# Autodesk Inventor assembly: liftpossible
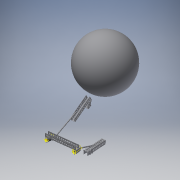
[picture p0: Inventor's stored thumbnail of the model, 180x180]
Saved by Autodesk Inventor 2016 (Build 200138000, 138)
## iProperties
Created: 2017-01-28
Part Number: liftpossible
Document SubType Name: Assembly
Designer: RoboticsUser
Author: RoboticsUser
## Documents named in this file (9)
- C:\Robotics\CAD\2016-17_CAD\liftpossible.iam
- C:\Robotics\CAD\2016-17_CAD\CapBall2.ipt
- C:\Robotics\CAD\COTSParts\Actobotics\585 parts\585450.ipt
- C:\Robotics\CAD\COTSParts\Actobotics\585 parts\585440.ipt
- C:\Robotics\CAD\COTSParts\Actobotics\585 parts\585404.ipt
- C:\Robotics\CAD\COTSParts\Actobotics\585 parts\585423.ipt
- C:\Robotics\CAD\COTSParts\Tetrix\Tetrix servo 180.ipt
- C:\Robotics\CAD\COTSParts\Tetrix\ptp_tetrix_servoframe_bracket.ipt
- C:\Robotics\CAD\COTSParts\Actobotics\585 parts\585454.ipt
## Components (20 placed, 8 different names)
1. CapBall2:1
2. 585450:1 — Insert:1, Insert:2, Insert:5, Insert:7, Insert:17
3. 585450:2 — Insert:9, Insert:10, Insert:11, Insert:12, Insert:18
4. 585440:1 — Insert:3, Insert:4, Insert:6, Insert:8
5. 585440:2 — Insert:13, Insert:14, Insert:15, Insert:16
6. 585404:1 — Insert:1, Insert:4
7. 585404:2 — Insert:2, Insert:3
8. 585423:1 — Insert:18, Insert:20
9. 585423:2 — Insert:17, Insert:19
10. 585404:3 — Insert:7, Insert:8
11. 585404:4 — Insert:5, Insert:6
12. 585404:5 — Insert:12, Insert:14
13. 585404:6 — Insert:9, Insert:15
14. 585404:7 — Insert:10, Insert:16
15. 585404:8 — Insert:11, Insert:13
16. Tetrix servo 180:1 — Insert:19, Mate:3, Mate:4, Flush:2
17. Tetrix servo 180:2 — Insert:20, Mate:1, Mate:2, Flush:1
18. ptp_tetrix_servoframe_bracket:1 — Mate:1, Mate:2, Flush:1, Mate:6, Flush:5, Flush:6
19. ptp_tetrix_servoframe_bracket:2 — Mate:3, Mate:4, Flush:2, Flush:3, Flush:4, Mate:5
20. 585454:1 — Flush:3, Flush:4, Mate:5, Mate:6, Flush:5, Flush:6
## Relationships (32: Insert 20, Mate 6, Flush 6)
- Insert:1: 585450:1 ↔ 585404:1
- Insert:2: 585450:1 ↔ 585404:2
- Insert:3: 585440:1 ↔ 585404:2
- Insert:4: 585440:1 ↔ 585404:1
- Insert:5: 585450:1 ↔ 585404:4
- Insert:6: 585440:1 ↔ 585404:4
- Insert:7: 585450:1 ↔ 585404:3
- Insert:8: 585440:1 ↔ 585404:3
- Insert:9: 585450:2 ↔ 585404:6
- Insert:10: 585450:2 ↔ 585404:7
- Insert:11: 585450:2 ↔ 585404:8
- Insert:12: 585450:2 ↔ 585404:5
- Insert:13: 585440:2 ↔ 585404:8
- Insert:14: 585440:2 ↔ 585404:5
- Insert:15: 585440:2 ↔ 585404:6
- Insert:16: 585440:2 ↔ 585404:7
- Insert:17: 585450:1 ↔ 585423:2
- Insert:18: 585450:2 ↔ 585423:1
- Insert:19: 585423:2 ↔ Tetrix servo 180:1
- Insert:20: 585423:1 ↔ Tetrix servo 180:2
- Mate:1: Tetrix servo 180:2 ↔ ptp_tetrix_servoframe_bracket:1
- Mate:2: Tetrix servo 180:2 ↔ ptp_tetrix_servoframe_bracket:1
- Flush:1: Tetrix servo 180:2 ↔ ptp_tetrix_servoframe_bracket:1
- Mate:3: Tetrix servo 180:1 ↔ ptp_tetrix_servoframe_bracket:2
- Mate:4: Tetrix servo 180:1 ↔ ptp_tetrix_servoframe_bracket:2
- Flush:2: Tetrix servo 180:1 ↔ ptp_tetrix_servoframe_bracket:2
- Flush:3: ptp_tetrix_servoframe_bracket:2 ↔ 585454:1
- Flush:4: ptp_tetrix_servoframe_bracket:2 ↔ 585454:1
- Mate:5: ptp_tetrix_servoframe_bracket:2 ↔ 585454:1
- Mate:6: ptp_tetrix_servoframe_bracket:1 ↔ 585454:1
- Flush:5: ptp_tetrix_servoframe_bracket:1 ↔ 585454:1
- Flush:6: ptp_tetrix_servoframe_bracket:1 ↔ 585454:1
